# Autodesk Inventor assembly: PULLEY ASSEMBLY
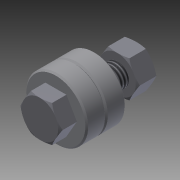
[picture p0: Inventor's stored thumbnail of the model, 180x180]
Saved by Autodesk Inventor 2013 (Build 170138000, 138)
## iProperties
Created: 2014-03-03
Part Number: PULLEY ASSEMBLY
Document SubType Name: Assembly
Designer: employee
Author: employee
## Documents named in this file (5)
- C:\Users\employee\Desktop\CoreXZ\PULLEY ASSEMBLY.iam
- C:\Users\employee\Desktop\CoreXZ\608.ipt
- C:\Users\employee\Desktop\CoreXZ\M8X30.ipt
- C:\Users\employee\Desktop\CoreXZ\M8 WASHER.ipt
- C:\Users\employee\Desktop\CoreXZ\M8 NUT.ipt
## Components (5 placed, 4 different names)
1. 608:1 — Insert:1, Insert:3
2. 608:2 — Insert:1, Insert:2
3. M8X30:1 — Insert:2
4. M8 WASHER:1 — Insert:3, Insert:4
5. M8 NUT:1 — Insert:4
## Relationships (4: Insert 4)
- Insert:1: 608:1 ↔ 608:2
- Insert:2: 608:2 ↔ M8X30:1
- Insert:3: 608:1 ↔ M8 WASHER:1
- Insert:4 (6.477 mm): M8 WASHER:1 ↔ M8 NUT:1
